# Autodesk Inventor assembly: CAR_011_VersaPlanetary_v2_Single_Stage_10_1_with_775_Series_Reverse_MIR
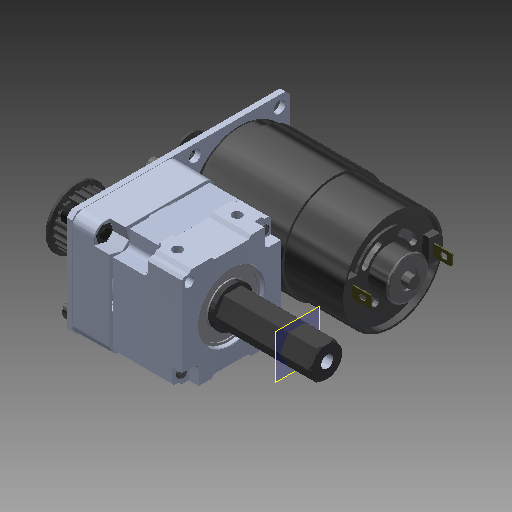
[picture p0: Inventor's stored thumbnail of the model, 512x512]
Saved by Autodesk Inventor 2018 (Build 220112000, 112)
## iProperties
Created: 2016-10-31
Part Number: CAR_011_VersaPlanetary_v2_Single_Stage_10_1_with_775_Series_Reverse_MIR
Description: STEP AP214
Document SubType Name: Assembly
Designer: user
Mass: 725.748 g
Surface Area: 818.614 cm^2
Volume: 178.454 cm^3
Density: 4.06686 g/cm^3
Title: 217-4973_1stage_775pro.STEP
Revision Number: ANY
Sending System: SolidWorks 2016
Preprocessor: SwSTEP 2.0
## Documents named in this file (16)
- C:\Users\user\Documents\GrabCAD\New folder\Build season\CAR_011_VersaPlanetary_v2_Single_Stage_10_1_with_775_Series_Reverse_MIR.iam
- C:\Users\user\Documents\GrabCAD\Deep Space 2019\Build Season\Vexpro Dump\217-2625-026 Rev1_MIR.ipt
- C:\Users\user\Documents\GrabCAD\Deep Space 2019\Build Season\Vexpro Dump\217-2742-001 Rev4_MIR.ipt
- C:\Users\user\Documents\GrabCAD\Deep Space 2019\Build Season\Vexpro Dump\217-2625-017 Rev1_9714K61_MIR.ipt
- C:\Users\user\Documents\GrabCAD\Deep Space 2019\Build Season\Vexpro Dump\217-2625-003 Rev1_MIR.ipt
- C:\Users\user\Documents\GrabCAD\Deep Space 2019\Build Season\Vexpro Dump\217-2625-018 Rev1_98541A410_MIR.ipt
- C:\Users\user\Documents\GrabCAD\Deep Space 2019\Build Season\Master references\832-1750-Ring-Gear-Screw_SSA0832-0500ZC_MIR.ipt
- C:\Users\user\Documents\GrabCAD\Deep Space 2019\Build Season\Vexpro Dump\217-4649-002 Rev1_SSA0832-0500ZC_MIR.ipt
- C:\Users\user\Documents\GrabCAD\Deep Space 2019\Build Season\Master references\217-4347-000 Rev1_MIR.ipt
- C:\Users\user\Documents\GrabCAD\Deep Space 2019\Build Season\Brainstorming\climber cad\217-2820 Rev1_Public_MIR2.iam
- C:\Users\user\Documents\GrabCAD\Deep Space 2019\Build Season\Master references\217-2816-001 Rev1_MIR.ipt
- C:\Users\user\Documents\GrabCAD\Deep Space 2019\Build Season\Vexpro Dump\217-4649-007 Rev1_94105A824_MIR.ipt
- C:\Users\user\Documents\GrabCAD\Deep Space 2019\Build Season\Master references\VersaPlanetary_180_Drive_-_Speed_Reducer_MIR.iam
- C:\Users\user\Documents\GrabCAD\Deep Space 2019\Build Season\Master references\VersaPlanetary_180_Drive_Gusset_Kit_MIR.ipt
- C:\Users\user\Documents\GrabCAD\Deep Space 2019\Build Season\Master references\12t_x_9mm_Wide_Double_Flange_Aluminum_Pulley_GT2_3mm_RS775_Motor_217-5871_MIR.ipt
- C:\Users\user\Documents\GrabCAD\Deep Space 2019\Build Season\Master references\24t_x_9mm_Wide_Double_Flange_Aluminum_Pulley_GT2_3mm_1_2_Hex_Bore_217-5875_MIR.ipt
## Components (18 placed, 15 different names)
1. 217-2625-026 Rev1_MIR:1
2. 217-2742-001 Rev4_MIR:1
3. 217-2742-001 Rev4_MIR:2
4. 217-2625-017 Rev1_9714K61_MIR:1
5. 217-2625-003 Rev1_MIR:1
6. 217-2625-018 Rev1_98541A410_MIR:1
7. 832-1750-Ring-Gear-Screw_SSA0832-0500ZC_MIR:1
8. 832-1750-Ring-Gear-Screw_SSA0832-0500ZC_MIR:2 — Mate:5
9. 217-4649-002 Rev1_SSA0832-0500ZC_MIR:1 — Insert:6
10. 217-4649-002 Rev1_SSA0832-0500ZC_MIR:2 — Mate:4, Insert:7
11. 217-4347-000 Rev1_MIR:1 — Insert:9, Mate:6
12. 217-2820 Rev1_Public_MIR2:1 [sub-assembly]
13. 217-2816-001 Rev1_MIR:1 — Insert:3
14. 217-4649-007 Rev1_94105A824_MIR:1
15. VersaPlanetary_180_Drive_-_Speed_Reducer_MIR:1 [sub-assembly] — Mate:5, Mate:4, Insert:3, Insert:4, Insert:8
16. VersaPlanetary_180_Drive_Gusset_Kit_MIR:1 — Insert:9, Insert:7, Insert:6, Insert:4
17. 12t_x_9mm_Wide_Double_Flange_Aluminum_Pulley_GT2_3mm_RS775_Motor_217-5871_MIR:1 — Mate:6, Flush:2
18. 24t_x_9mm_Wide_Double_Flange_Aluminum_Pulley_GT2_3mm_1_2_Hex_Bore_217-5875_MIR:1 — Flush:2, Insert:8
## Relationships (10: Insert 6, Mate 3, Flush 1)
- Mate:5: 832-1750-Ring-Gear-Screw_SSA0832-0500ZC_MIR:2 ↔ VersaPlanetary_180_Drive_-_Speed_Reducer_MIR:1
- Mate:4: 217-4649-002 Rev1_SSA0832-0500ZC_MIR:2 ↔ VersaPlanetary_180_Drive_-_Speed_Reducer_MIR:1
- Insert:3: 217-2816-001 Rev1_MIR:1 ↔ VersaPlanetary_180_Drive_-_Speed_Reducer_MIR:1
- Insert:9: 217-4347-000 Rev1_MIR:1 ↔ VersaPlanetary_180_Drive_Gusset_Kit_MIR:1
- Insert:7: 217-4649-002 Rev1_SSA0832-0500ZC_MIR:2 ↔ VersaPlanetary_180_Drive_Gusset_Kit_MIR:1
- Insert:6: 217-4649-002 Rev1_SSA0832-0500ZC_MIR:1 ↔ VersaPlanetary_180_Drive_Gusset_Kit_MIR:1
- Insert:4: VersaPlanetary_180_Drive_-_Speed_Reducer_MIR:1 ↔ VersaPlanetary_180_Drive_Gusset_Kit_MIR:1
- Mate:6: 217-4347-000 Rev1_MIR:1 ↔ 12t_x_9mm_Wide_Double_Flange_Aluminum_Pulley_GT2_3mm_RS775_Motor_217-5871_MIR:1
- Flush:2: 12t_x_9mm_Wide_Double_Flange_Aluminum_Pulley_GT2_3mm_RS775_Motor_217-5871_MIR:1 ↔ 24t_x_9mm_Wide_Double_Flange_Aluminum_Pulley_GT2_3mm_1_2_Hex_Bore_217-5875_MIR:1
- Insert:8: VersaPlanetary_180_Drive_-_Speed_Reducer_MIR:1 ↔ 24t_x_9mm_Wide_Double_Flange_Aluminum_Pulley_GT2_3mm_1_2_Hex_Bore_217-5875_MIR:1
